# Autodesk Inventor assembly: ASY MSC 010 cone
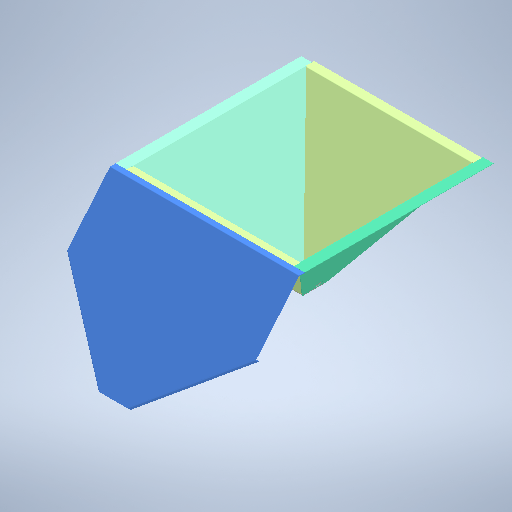
[picture p0: Inventor's stored thumbnail of the model, 512x512]
Saved by Autodesk Inventor 2025 (Build 290162010, 162A)
## iProperties
Created: 2024-05-19
Part Number: ASY MSC 010 cone
Document SubType Name: Assembly
Designer: admin
Mass: 24706.5 g
Surface Area: 124528 cm^2
Volume: 24706.5 cm^3
Density: 1 g/cm^3
Stock Number: ASY МОО 010 конус
Author: admin
## Documents named in this file (8)
- C:\Users\pokla\Documents\Inventor\Отстойник осветлитель\Manturovo_Se-clar-Gleb\ASY MSC 010 cone.iam
- C:\Users\pokla\Documents\Inventor\Отстойник осветлитель\Manturovo_Se-clar-Gleb\конус\MSC 014 cone IN right board.ipt
- C:\Users\pokla\Documents\Inventor\Отстойник осветлитель\Manturovo_Se-clar-Gleb\конус\MSC 011 cone IN bottom.ipt
- C:\Users\pokla\Documents\Inventor\Отстойник осветлитель\Manturovo_Se-clar-Gleb\конус\MSC 013 cone IN left board.ipt
- C:\Users\pokla\Documents\Inventor\Отстойник осветлитель\Manturovo_Se-clar-Gleb\конус\MSC 012 cone IN back.ipt
- C:\Users\pokla\Documents\Inventor\Отстойник осветлитель\Manturovo_Se-clar-Gleb\конус\MSC 019 cone sketch.ipt
- C:\Users\pokla\Documents\Inventor\Отстойник осветлитель\Manturovo_Se-clar-Gleb\конус\MSC 015 cone IN bow.ipt
- C:\Users\pokla\Documents\Inventor\Отстойник осветлитель\Manturovo_Se-clar-Gleb\конус\MSC 016 cone exit back.ipt
## Components (7 placed, 7 different names)
1. МОО 019 конус эскиз:1 — Flush:8, Flush:9, Mate:1
2. МОО 022 конус подача корма — Flush:6, Flush:10, Mate:2, Flush:12
3. МОО 011 конус подача дно:1 — Flush:4, Flush:5, Flush:11
4. МОО 014 конус подача правый борт:1 — Rigid:3, Flush:12, Flush:13
5. МОО 013 конус подача левый борт:1 — Mate:4, Flush:14, Mate:5
6. МОО 015 конус подача нос:1 — Rigid:3, Rigid:8, Mate:3
7. МОО 016 конус выход корма:1 — Rigid:8
## Relationships (17: Flush 10, Mate 5, WeldJoint 2)
- Flush:4: МОО 011 конус подача дно:1
- Flush:5: МОО 011 конус подача дно:1
- Flush:6: МОО 022 конус подача корма
- Flush:8: МОО 019 конус эскиз:1
- Flush:9: МОО 019 конус эскиз:1
- Mate:1: МОО 019 конус эскиз:1
- Flush:10: МОО 022 конус подача корма
- Mate:2: МОО 022 конус подача корма
- Flush:11 (-230 mm): МОО 011 конус подача дно:1
- Rigid:3 [WeldJoint]: МОО 014 конус подача правый борт:1 ↔ МОО 015 конус подача нос:1
- Rigid:8 [WeldJoint]: МОО 015 конус подача нос:1 ↔ МОО 016 конус выход корма:1
- Mate:3: МОО 015 конус подача нос:1
- Flush:12: МОО 022 конус подача корма ↔ МОО 014 конус подача правый борт:1
- Flush:13: МОО 014 конус подача правый борт:1
- Mate:4: МОО 013 конус подача левый борт:1
- Flush:14: МОО 013 конус подача левый борт:1
- Mate:5: МОО 013 конус подача левый борт:1
